# Autodesk Inventor assembly: frame
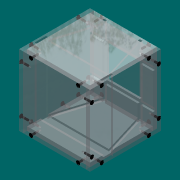
[picture p0: Inventor's stored thumbnail of the model, 180x180]
Saved by Autodesk Inventor 2016 (Build 200138000, 138)
## iProperties
Created: 2015-10-13
Part Number: frame
Document SubType Name: Assembly
Designer: Sawaiz
Author: Sawaiz
## Documents named in this file (7)
- C:\Users\Sawaiz\OneDrive\projects\modularRICH\frame\frame.iam
- C:\Users\Sawaiz\OneDrive\projects\modularRICH\frame\front.ipt
- C:\Users\Sawaiz\OneDrive\projects\modularRICH\frame\sides.ipt
- C:\Users\Sawaiz\OneDrive\projects\modularRICH\frame\topBottom.ipt
- C:\Users\Sawaiz\OneDrive\projects\modularRICH\frame\back.ipt
- C:\Users\Sawaiz\OneDrive\projects\modularRICH\frame\m3x12Flat.ipt
- C:\Users\Sawaiz\OneDrive\projects\modularRICH\modularRICH.xlsx
## Components (31 placed, 5 different names)
1. front:1 — Flush:2, Flush:4, Mate:1, Mate:6, Flush:13, Mate:23, Mate:24, Angle:10, Angle:11
2. sides:1 — Flush:11, Mate:9, Flush:12, Flush:13, Mate:15, Angle:2, Mate:16, Angle:3, Mate:17, Angle:4, Mate:18, Angle:5
3. sides:2 — Flush:2, Flush:4, Mate:1, Flush:5, Flush:8, Mate:7, Mate:10, Mate:19, Mate:20, Mate:21, Mate:22, Angle:6, Angle:7, Angle:8, Angle:9
4. topBottom:1 — Flush:5, Mate:6, Mate:7
5. topBottom:2 — Flush:9, Flush:10, Mate:8, Flush:11, Mate:9, Mate:10
6. back:1 — Flush:8, Flush:9, Flush:10, Mate:8, Flush:12, Mate:11, Mate:12, Mate:13, Mate:14, Angle:1
7. m3x12Flat:1 — Mate:11, Mate:12, Mate:13
8. m3x12Flat:2
9. m3x12Flat:3 — Mate:14, Angle:1
10. m3x12Flat:4
11. m3x12Flat:5 — Mate:15, Angle:2
12. m3x12Flat:6
13. m3x12Flat:7 — Mate:16, Angle:3
14. m3x12Flat:8
15. m3x12Flat:9 — Mate:17, Angle:4
16. m3x12Flat:10
17. m3x12Flat:11 — Mate:18, Angle:5
18. m3x12Flat:12
19. m3x12Flat:13 — Mate:19, Angle:7
20. m3x12Flat:17
21. m3x12Flat:15 — Mate:21, Angle:9
22. m3x12Flat:18
23. m3x12Flat:19
24. m3x12Flat:14 — Mate:20, Angle:8
25. m3x12Flat:20
26. m3x12Flat:16 — Mate:22, Angle:6
27. m3x12Flat:21
28. m3x12Flat:22 — Mate:23, Angle:11
29. m3x12Flat:24
30. m3x12Flat:23 — Mate:24, Angle:10
31. m3x12Flat:25
## Component patterns: (4 elements, first: m3x12Flat:1), (4 elements, first: m3x12Flat:3), (4 elements, first: m3x12Flat:5), (4 elements, first: m3x12Flat:7), (4 elements, first: m3x12Flat:9), (4 elements, first: m3x12Flat:11), (4 elements, first: m3x12Flat:13), (4 elements, first: m3x12Flat:15), (4 elements, first: m3x12Flat:14), (4 elements, first: m3x12Flat:16), (4 elements, first: m3x12Flat:22), (4 elements, first: m3x12Flat:23)
## Relationships (40: Mate 20, Angle 11, Flush 9)
- Flush:2: front:1 ↔ sides:2
- Flush:4: front:1 ↔ sides:2
- Mate:1: front:1 ↔ sides:2
- Flush:5: sides:2 ↔ topBottom:1
- Flush:8: sides:2 ↔ back:1
- Mate:6: front:1 ↔ topBottom:1
- Mate:7: sides:2 ↔ topBottom:1
- Flush:9: topBottom:2 ↔ back:1
- Flush:10: topBottom:2 ↔ back:1
- Mate:8: topBottom:2 ↔ back:1
- Flush:11: sides:1 ↔ topBottom:2
- Mate:9: sides:1 ↔ topBottom:2
- Mate:10: sides:2 ↔ topBottom:2
- Flush:12: sides:1 ↔ back:1
- Flush:13: front:1 ↔ sides:1
- Mate:11: back:1 ↔ m3x12Flat:1
- Mate:12: back:1 ↔ m3x12Flat:1
- Mate:13: back:1 ↔ m3x12Flat:1
- Mate:14: back:1 ↔ m3x12Flat:3
- Angle:1 (0 deg): back:1 ↔ m3x12Flat:3
- Mate:15: sides:1 ↔ m3x12Flat:5
- Angle:2 (0 deg): sides:1 ↔ m3x12Flat:5
- Mate:16: sides:1 ↔ m3x12Flat:7
- Angle:3 (0 deg): sides:1 ↔ m3x12Flat:7
- Mate:17: sides:1 ↔ m3x12Flat:9
- Angle:4 (0 deg): sides:1 ↔ m3x12Flat:9
- Mate:18: sides:1 ↔ m3x12Flat:11
- Angle:5 (0 deg): sides:1 ↔ m3x12Flat:11
- Mate:19: sides:2 ↔ m3x12Flat:13
- Mate:20: sides:2 ↔ m3x12Flat:14
- Mate:21: sides:2 ↔ m3x12Flat:15
- Mate:22: sides:2 ↔ m3x12Flat:16
- Angle:6 (0 deg): sides:2 ↔ m3x12Flat:16
- Angle:7 (0 deg): sides:2 ↔ m3x12Flat:13
- Angle:8 (0 deg): sides:2 ↔ m3x12Flat:14
- Angle:9 (0 deg): sides:2 ↔ m3x12Flat:15
- Mate:23: front:1 ↔ m3x12Flat:22
- Mate:24: front:1 ↔ m3x12Flat:23
- Angle:10 (0 deg): front:1 ↔ m3x12Flat:23
- Angle:11 (0 deg): front:1 ↔ m3x12Flat:22
## Named parameters: acrylicThickness = 6.35 mm, aerogelThickness = 20 mm, height = 100 mm, width = 100 mm, depth = 100 mm, mirrorAngle = 17 deg, detectorWidth = 52 mm, detectorHeight = 52 mm, mirrorThickness = 3 mm, fresnelThickness = 0.1 mm, grooveDensity = 100, focalLength = 76.2 mm, ior = 1.49, centerThickness = 1.524 mm, fresnelAngle = 90 deg, fresnelEffectiveDiameter = 76.2 mm, mirrorSuppourtWidth = 40 mm
